# Autodesk Inventor assembly: antenna_assembled
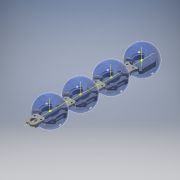
[picture p0: Inventor's stored thumbnail of the model, 180x180]
Saved by Autodesk Inventor 2017 (Build 210142000, 142)
## iProperties
Created: 2018-05-30
Part Number: antenna_assembled
Document SubType Name: Assembly
Designer: Nic
Author: Nic
## Documents named in this file (6)
- C:\Users\Nic\Documents\Antenna\antenna_assembled.iam
- C:\Users\Nic\Documents\Antenna\top_segment.ipt
- C:\Users\Nic\Documents\Antenna\sleeve.ipt
- C:\Users\Nic\Documents\Antenna\rod.ipt
- C:\Users\Nic\Documents\Antenna\middle_segment.ipt
- C:\Users\Nic\Documents\Antenna\sensor_pad.ipt
## Components (14 placed, 5 different names)
1. top_segment:1 — Insert:13, Insert:14, Angle:3
2. sleeve:1 — Insert:13
3. rod:1 — Insert:12
4. middle_segment:1 — Insert:4, Insert:12, Insert:14, Insert:15, Angle:2, Angle:3, Mate:3, Mate:5, Ball:1
5. sleeve:2 — Insert:4, Insert:5
6. rod:2 — Insert:5
7. middle_segment:2 — Insert:7, Insert:15, Insert:9, Angle:1, Angle:2, Mate:7, Ball:2
8. sensor_pad:1 — Mate:2
9. sensor_pad:2 — Mate:4, Ball:1
10. sensor_pad:3 — Mate:6, Ball:2
11. middle_segment:3 — Insert:9, Angle:1, Mate:8, Ball:3
12. sleeve:3 — Insert:7, Insert:8
13. rod:3 — Insert:8
14. sensor_pad:4 — Mate:1, Ball:3
## Relationships (23: Insert 9, Mate 8, Angle 3, BallJoint 3)
- Insert:4: middle_segment:1 ↔ sleeve:2
- Insert:5: sleeve:2 ↔ rod:2
- Insert:7: middle_segment:2 ↔ sleeve:3
- Insert:8: sleeve:3 ↔ rod:3
- Insert:9: middle_segment:2 ↔ middle_segment:3
- Insert:12: rod:1 ↔ middle_segment:1
- Insert:13: top_segment:1 ↔ sleeve:1
- Insert:14: top_segment:1 ↔ middle_segment:1
- Insert:15: middle_segment:1 ↔ middle_segment:2
- Angle:1 (0 deg): middle_segment:2 ↔ middle_segment:3
- Angle:2 (0 deg): middle_segment:1 ↔ middle_segment:2
- Angle:3 (0 deg): top_segment:1 ↔ middle_segment:1
- Mate:1: sensor_pad:4
- Mate:2: sensor_pad:1
- Mate:3: middle_segment:1
- Mate:4: sensor_pad:2
- Mate:5: middle_segment:1
- Mate:6: sensor_pad:3
- Mate:7: middle_segment:2
- Mate:8: middle_segment:3
- Ball:1: middle_segment:1 ↔ sensor_pad:2
- Ball:2: middle_segment:2 ↔ sensor_pad:3
- Ball:3: middle_segment:3 ↔ sensor_pad:4
